# Autodesk Inventor assembly: 6inch_mirror
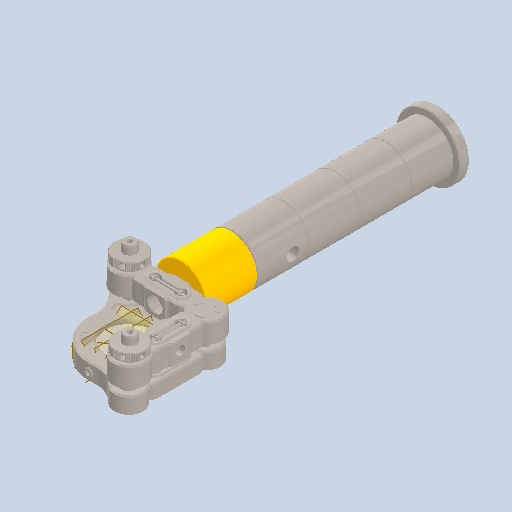
[picture p0: Inventor's stored thumbnail of the model, 512x512]
Saved by Autodesk Inventor 2026.1 (Build 301233000, 233)
## iProperties
Created: 2019-05-27
Part Number: 6inch_mirror
Document SubType Name: Assembly
Designer: Julian
Author: Julian
## Documents named in this file (5)
- C:\Users\user\Desktop\setup_inventor_2025\LightPath\6 inch mirrors\6inch_mirror.iam
- C:\Users\user\Desktop\setup_inventor_2025\LightPath\6 inch mirrors\M-PS-4_4in_ped_post.ipt
- C:\Users\user\Desktop\setup_inventor_2025\LightPath\bridge final\M-PS-1E_1in_post.ipt
- C:\Users\user\Desktop\setup_inventor_2025\LightPath\bridge final\SS100-F2H_suprema_1in_mirror_mount.ipt
- C:\Users\user\Desktop\setup_inventor_2025\LightPath\bridge final\1in_5mm_mir.ipt
## Components (4 placed, 4 different names)
1. M-PS-4_4in_ped_post:1 — Passend:3, Passend:4
2. M-PS-1E_1in_post:1 — Passend:3, Passend:4, Passend:5, Passend:6
3. SS100-F2H_suprema_1in_mirror_mount:1 — Passend:1, Passend:2, Passend:5, Passend:6
4. 1in_5mm_mir:1 — Passend:1, Passend:2
## Relationships (6: Mate 6)
- Passend:1 [Mate]: SS100-F2H_suprema_1in_mirror_mount:1 ↔ 1in_5mm_mir:1
- Passend:2 [Mate]: SS100-F2H_suprema_1in_mirror_mount:1 ↔ 1in_5mm_mir:1
- Passend:3 [Mate]: M-PS-4_4in_ped_post:1 ↔ M-PS-1E_1in_post:1
- Passend:4 [Mate]: M-PS-4_4in_ped_post:1 ↔ M-PS-1E_1in_post:1
- Passend:5 [Mate]: M-PS-1E_1in_post:1 ↔ SS100-F2H_suprema_1in_mirror_mount:1
- Passend:6 [Mate]: M-PS-1E_1in_post:1 ↔ SS100-F2H_suprema_1in_mirror_mount:1
